# Autodesk Inventor assembly: SZ045F-16-018-27
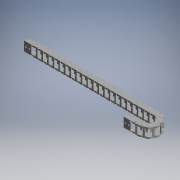
[picture p0: Inventor's stored thumbnail of the model, 180x180]
Saved by Autodesk Inventor 2017.3 (Build 213256000, 256)
## iProperties
Category: PARTsolutions
Company: MISUMI
Part Number: SZ045F-16-018-27
Catalog Web Link: www.cadenas.de
Description: SE045F-_ _, SZ045F-_ _, SE08F-_ _, SZ08F-_ _, SE14F-_, SZ14F-_, SE16F-_, SZ16F-_, SE200F-_ _,SZ200F-_ _, SE300F-_ _,SZ300F-_ _-Cable Carriers - Link Number Specified Type - Flanged
Vendor: MISUMI
Document SubType Name: Assembly
Designer: partserver
Manufacturer: MISUMI
Mass: 36.3529 g
Surface Area: 524.597 cm^2
Volume: 36.3529 cm^3
Density: 1 g/cm^3
Title: SZ045F-16-018-27
Author: Cadenas PARTsolutions
Comments: Cable Carriers - Link Number Specified Type - Flanged
PSOL_IDENT_0: {$CADENAS_DATA\23d-libs\misumi\metric\07_slide_rails\se08f_asmtab.prj},315 {VTYP=3D},{STYP=ASSTAB},{
PSOL_IDENT_1: NB=SZ045F-16-018-27},{LINA=SZ045F-16-018-27},{NN=SE045F-_ _, SZ045F-_ _, SE08F-_ _, SZ08F-_ _, SE14F
PSOL_IDENT_2: -_, SZ14F-_, SE16F-_, SZ16F-_, SE200F-_ _,SZ200F-_ _, SE300F-_ _,SZ300F-_ _},{DATE=30.06.2021 12:54:
PSOL_IDENT_3: 06},{GEOMDATE=08.06.2010},{VERSION=},{LINEID=10},{WBVAR=TYS,NO,R,NOL},{WBNUMERIC=NO,NOL}  {NB=SZ045F
PSOL_IDENT_4: -16-018-27},{LINA=SZ045F-16-018-27},{KT=DUMMY},{PN=SZ045F-16-018-27},{TYPE=SZ045F},{TYS=2},{TYSCONF=
PSOL_IDENT_5: 045},{TS=SZ045F},{TSCONF1= '1','For Free End', '2','For Fixed End' },{TSCONFH=1},{TSCONFP=2},{MAT=Sp
PSOL_IDENT_6: ecial Plastic},{OT=-30~100},{NO=16},{NO0=16},{R=018},{BR0='018','028','038'},{R1=18},{NOL=27},{NOL1=
PSOL_IDENT_7: [1:27]},{H=50},{H1=37.5},{HF=60},{K=95},{P=13},{B=13},{LL=22},{A=9.4},{C=16},{C2=16},{D=-},{E=-},{W=
PSOL_IDENT_8: 23.0},{F=-},{G=22},{NCT=-},{WL=1.4},{AFFREE=045-16-1},{AFFIX=045-16-2},{DD=50},{PP=13.0},{HH=12.5},{
PSOL_IDENT_9: N=4},{XALG=1.818019},{HB=19.5},{HB1=19.5},{X=22.3},{PPATH=se200f/se08f_asmtpl.prj}
NB: SZ045F-16-018-27
NN: SE045F-_ _, SZ045F-_ _, SE08F-_ _, SZ08F-_ _, SE14F-_, SZ14F-_, SE16F-_, SZ16F-_, SE200F-_ _,SZ200F-_ _, SE300F-_ _,SZ300F-_ _
NT: Cable Carriers - Link Number Specified Type - Flanged
NBSYN: $PN.
LINA: SZ045F-16-018-27
CATALOG: Misumi
PN: SZ045F-16-018-27
TYS: Inner Radius Mount
TS: SZ045F
MAT: Special Plastic
OT: -30~100
NO: 16
R: 018
NOL: 27
H: 50
H1: 37.5
HF: 60
K: 95
P: 13
B: 13
LL: 22
A: 9.4
C: 16
D: -
E: -
W: 23
F: -
G: 22
NCT: -
WL: 1.4
SUPPLIER: MISUMI
ARTICLENO: SZ045F-16-018-27
BOMINFO: SZ045F-16-018-27
CREATOR: CADENAS GmbH
## Documents named in this file (4)
- e:\temp\worker_7\temp\exporttempdir_636_80_eg8Pk\format_0\SZ045F-16-018-27.iam
- e:\temp\worker_7\temp\exporttempdir_636_80_eg8Pk\format_0\SZ045F-16-018-27c.ipt
- e:\temp\worker_7\temp\exporttempdir_636_80_eg8Pk\format_0\045-16-1_se08f.ipt
- e:\temp\worker_7\temp\exporttempdir_636_80_eg8Pk\format_0\045-16-2_se08f.ipt
## Components (29 placed, 3 different names)
1. SZ045F-16-018-27c:1 — move_2_XY@1 <-> move_1_XY@2, move_2_Z@1 <-> move_1_Z@2, move_1_XY@1 <-> end_2_XY@7, move_1_Z@1 <-> end_2_Z@7
2. SZ045F-16-018-27c:2 — move_2_XY@1 <-> move_1_XY@2, move_2_Z@1 <-> move_1_Z@2, move_2_XY@2 <-> move_1_XY@3, move_2_Z@2 <-> move_1_Z@3
3. SZ045F-16-018-27c:3 — move_2_XY@2 <-> move_1_XY@3, move_2_Z@2 <-> move_1_Z@3, move_2_XY@3 <-> move_1_XY@4, move_2_Z@3 <-> move_1_Z@4
4. SZ045F-16-018-27c:4 — move_2_XY@3 <-> move_1_XY@4, move_2_Z@3 <-> move_1_Z@4, move_2_XY@4 <-> move_1_XY@5, move_2_Z@4 <-> move_1_Z@5
5. SZ045F-16-018-27c:5 — move_2_XY@4 <-> move_1_XY@5, move_2_Z@4 <-> move_1_Z@5, move_2_XY@5 <-> move_1_XY@6, move_2_Z@5 <-> move_1_Z@6
6. SZ045F-16-018-27c:6 — move_2_XY@5 <-> move_1_XY@6, move_2_Z@5 <-> move_1_Z@6
7. 045-16-1_se08f:1 — move_1_XY@1 <-> end_2_XY@7, move_1_Z@1 <-> end_2_Z@7
8. SZ045F-16-018-27c:7
9. SZ045F-16-018-27c:8
10. SZ045F-16-018-27c:9
11. SZ045F-16-018-27c:10
12. SZ045F-16-018-27c:11
13. SZ045F-16-018-27c:12
14. SZ045F-16-018-27c:13
15. SZ045F-16-018-27c:14
16. SZ045F-16-018-27c:15
17. SZ045F-16-018-27c:16
18. SZ045F-16-018-27c:17
19. SZ045F-16-018-27c:18
20. SZ045F-16-018-27c:19
21. SZ045F-16-018-27c:20
22. SZ045F-16-018-27c:21
23. SZ045F-16-018-27c:22
24. SZ045F-16-018-27c:23
25. SZ045F-16-018-27c:24
26. SZ045F-16-018-27c:25
27. SZ045F-16-018-27c:26
28. SZ045F-16-018-27c:27
29. 045-16-2_se08f:1
## Relationships (12: Flush 6, Mate 6)
- move_2_XY@1 <-> move_1_XY@2 [Flush]: SZ045F-16-018-27c:1 ↔ SZ045F-16-018-27c:2
- move_2_Z@1 <-> move_1_Z@2 [Mate]: SZ045F-16-018-27c:1 ↔ SZ045F-16-018-27c:2
- move_2_XY@2 <-> move_1_XY@3 [Flush]: SZ045F-16-018-27c:2 ↔ SZ045F-16-018-27c:3
- move_2_Z@2 <-> move_1_Z@3 [Mate]: SZ045F-16-018-27c:2 ↔ SZ045F-16-018-27c:3
- move_2_XY@3 <-> move_1_XY@4 [Flush]: SZ045F-16-018-27c:3 ↔ SZ045F-16-018-27c:4
- move_2_Z@3 <-> move_1_Z@4 [Mate]: SZ045F-16-018-27c:3 ↔ SZ045F-16-018-27c:4
- move_2_XY@4 <-> move_1_XY@5 [Flush]: SZ045F-16-018-27c:4 ↔ SZ045F-16-018-27c:5
- move_2_Z@4 <-> move_1_Z@5 [Mate]: SZ045F-16-018-27c:4 ↔ SZ045F-16-018-27c:5
- move_2_XY@5 <-> move_1_XY@6 [Flush]: SZ045F-16-018-27c:5 ↔ SZ045F-16-018-27c:6
- move_2_Z@5 <-> move_1_Z@6 [Mate]: SZ045F-16-018-27c:5 ↔ SZ045F-16-018-27c:6
- move_1_XY@1 <-> end_2_XY@7 [Flush] (-1 mm): SZ045F-16-018-27c:1 ↔ 045-16-1_se08f:1
- move_1_Z@1 <-> end_2_Z@7 [Mate]: SZ045F-16-018-27c:1 ↔ 045-16-1_se08f:1
